# Autodesk Inventor assembly: USB_Assem_Sleeve_Answer
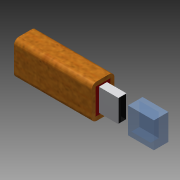
[picture p0: Inventor's stored thumbnail of the model, 180x180]
Saved by Autodesk Inventor 2015 (Build 190159000, 159)
## iProperties
Created: 2015-02-01
Part Number: USB_Assem_Sleeve_Answer
Document SubType Name: Assembly
Designer: Paul
Author: Paul
## Documents named in this file (4)
- C:\Users\paul\Google Drive\All #ResBaz Shared\Paul2AlizaCAD\06_Assembly\01_USB_Assembly\USB_Assem_Sleeve_Answer.iam
- C:\Users\paul\Google Drive\All #ResBaz Shared\Paul2AlizaCAD\06_Assembly\01_USB_Assembly\USB_Stick.ipt
- C:\Users\paul\Google Drive\All #ResBaz Shared\Paul2AlizaCAD\06_Assembly\01_USB_Assembly\USB_Cap.ipt
- C:\Users\paul\Google Drive\All #ResBaz Shared\Paul2AlizaCAD\06_Assembly\01_USB_Assembly\Sleeve.ipt
## Components (3 placed, 3 different names)
1. USB_Stick:1 — Flush:1, Flush:2, Mate:1, Mate:2, Mate:3, Flush:3
2. USB_Cap:1 — Flush:1, Flush:2, Mate:1
3. Sleeve:1 — Mate:2, Mate:3, Flush:3
## Relationships (6: Flush 3, Mate 3)
- Flush:1: USB_Stick:1 ↔ USB_Cap:1
- Flush:2: USB_Stick:1 ↔ USB_Cap:1
- Mate:1 (20 mm): USB_Stick:1 ↔ USB_Cap:1
- Mate:2: USB_Stick:1 ↔ Sleeve:1
- Mate:3: USB_Stick:1 ↔ Sleeve:1
- Flush:3: USB_Stick:1 ↔ Sleeve:1
